# Autodesk Inventor assembly: BNT 2010-2.6 +1166L C7T-J1K_10000KBK 15BF 15
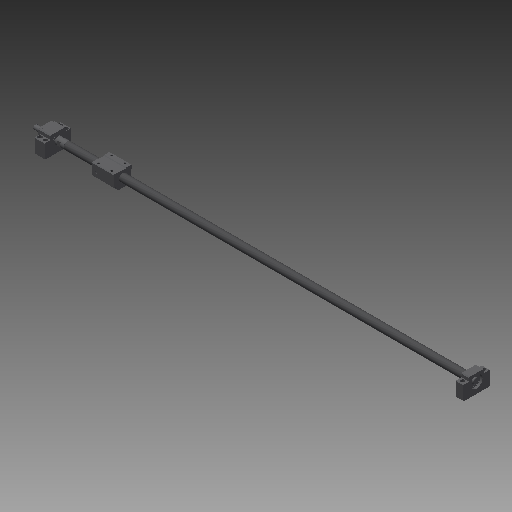
[picture p0: Inventor's stored thumbnail of the model, 512x512]
Saved by Autodesk Inventor 2018 (Build 220112000, 112)
## iProperties
Category: PARTsolutions
Company: THK
Created: 2017-05-30
Part Number: BNT 2010-2.6 +1166L C7T-J1K_10000KBK 15BF 15
Catalog Web Link: www.cadenas.de
Description: Rectangular-Nut Non-Preloaded Type BNT-
Vendor: THK
Document SubType Name: Assembly
Designer: psAdmin
Manufacturer: THK
PSOL_IDENT_0: {$CADENAS_DATA\23d-libs\thk\fed_screw\ball_screw\ball_screw\standard_lead_rbs\bnt_asmtab.prj},284 {V
PSOL_IDENT_1: TYP=3D},{STYP=ASSTAB},{NB=BNT 2010-2.6 +1166L C7T-J1K_10000KBK 15BF 15},{LINA=BNT 2010-2.6 +1166L C7
PSOL_IDENT_2: T-J1K},{NN=Rectangular-Nut Non-Preloaded Type BNT},{DATE=16.05.2017 06:09:49},{GEOMDATE=15.05.2017 0
PSOL_IDENT_3: 2:25:45},{VERSION=},{LINEID=490},{LINESUBID=-1},{WBVAR=TS,ST,FS,FSS,SS,SSS,A,PN}  {NB=BNT 2010-2.6 +
PSOL_IDENT_4: 1166L C7T-J1K_10000KBK 15BF 15},{LINA=BNT 2010-2.6 +1166L C7T-J1K},{KT=DUMMY},{TP=BNT series},{MN=BN
PSOL_IDENT_5: T 2010-2.6},{TS=},{ST=1000},{NOTE1=There is the groove on both ends of the stroke.},{FS=-J1},{FSS=BK
PSOL_IDENT_6: 15},{INFO1=Infotext},{SS=K},{SSS=BF 15},{INFO2=Infotext},{OL=1166},{NOTE2=Overall thread lenght is
PSOL_IDENT_7: added to the both ends of the stroke 10mm.},{A=C7},{PN=0},{C7=2000.000},{C8=2200.000},{C10=2200.000}
PSOL_IDENT_8: ,{FSX='','None','-H1','Type_H1','-H2','Type_H2','-H3','Type_H3','-J1','Type_J1','-J2','Type_J2','-J3'
PSOL_IDENT_9: ,'Type_J3'},{E3=13},{E4=13},{F1=20},{E1=40},{N1=6},{H1=9},{F2=20},{E2=49},{N2=6},{H2=9},{SD=20},{STX=
PSOL_IDENT_10: 2034},{EL=2092},{L=58},{FSX1=75},{SSX1=13},{AX1='C7','C7','C8','C8','','C10'},{PNX=500},{SS1=K},{PPA
PSOL_IDENT_11: TH=bnt/bnt_asmtpl.prj},{INFO1X=fixed_},{INFO2X=supported_},{FSSX='','None','BK 15','BK 15 (Rectangul
PSOL_IDENT_12: ar Type)'},{SSSX='','None','FF 15','FF 15 (Fixed side, Round Type)','EF 15','EF 15 (Rectangular Type
PSOL_IDENT_13: )','BF 15','BF 15 (Fixed side, Rectangular Type)'}
NN: Rectangular-Nut Non-Preloaded Type BNT
NB: BNT 2010-2.6 +1166L C7T-J1K_10000KBK 15BF 15
NBSYN: $MN. $TS.+$OL.L $A.T$FS.$SS1._$ST.$PN.$SS.$FSS.$SSS.
LINA: BNT 2010-2.6 +1166L C7T-J1K
MN: BNT 2010-2.6
TS: Without seal
ST: 1000
NOTE1: There is the groove on both ends of the stroke.
FS: Type_J1
FSS: BK 15 (Rectangular Type)
INFO1: Infotext
SS: Type_K
SSS: BF 15 (Rectangular Type)
INFO2: Infotext
OL: 1166.000
NOTE2: Overall thread lenght is added to the both ends of the stroke 10mm.
A: C7
PN: 0
SUPPLIER: THK
ARTICLENO: BNT 2010-2.6 +1166L C7T-J1K_10000KBK 15BF 15
BOMINFO: BNT 2010-2.6 +1166L C7T-J1K
CREATOR: CADENAS GmbH
Title: BNT 2010-2.6 +1166L C7T-J1K
Author: Cadenas PARTsolutions
## Documents named in this file (7)
- C:\Users\P301319\Documents\GitHub\CNC-Lathe-CAD\CNC Lathe Project\Project Files\AIS2016\BNT 2010-2_6 +1166L C7T-J1K_10000KBK 15BF 15.iam
- C:\Users\P301319\Documents\GitHub\CNC-Lathe-CAD\CNC Lathe Project\Project Files\AIS2016\BNT 2010-2_61000-J1K Shaft.ipt
- C:\Users\P301319\Documents\GitHub\CNC-Lathe-CAD\CNC Lathe Project\Project Files\AIS2016\BNT 2010-2_6 Nut.ipt
- C:\Users\P301319\Documents\GitHub\CNC-Lathe-CAD\CNC Lathe Project\Project Files\AIS2016\BK 15.ipt
- C:\Users\P301319\Documents\GitHub\CNC-Lathe-CAD\CNC Lathe Project\Project Files\AIS2016\BK 15collar.ipt
- C:\Users\P301319\Documents\GitHub\CNC-Lathe-CAD\CNC Lathe Project\Project Files\AIS2016\BF 15 Part2.ipt
- C:\Users\P301319\Documents\GitHub\CNC-Lathe-CAD\CNC Lathe Project\Project Files\AIS2016\BF 15 Part1.ipt
## Components (6 placed, 6 different names)
1. BNT 2010-2_61000-J1K Shaft:1 — Mate:1
2. BNT 2010-2_6 Nut:1 — Mate:1
3. BK 15:1
4. BK 15collar:1
5. BF 15 Part2:1
6. BF 15 Part1:1
## Relationships (1: Mate 1)
- Mate:1: BNT 2010-2_61000-J1K Shaft:1 ↔ BNT 2010-2_6 Nut:1
